# Autodesk Inventor assembly: dtandcata2
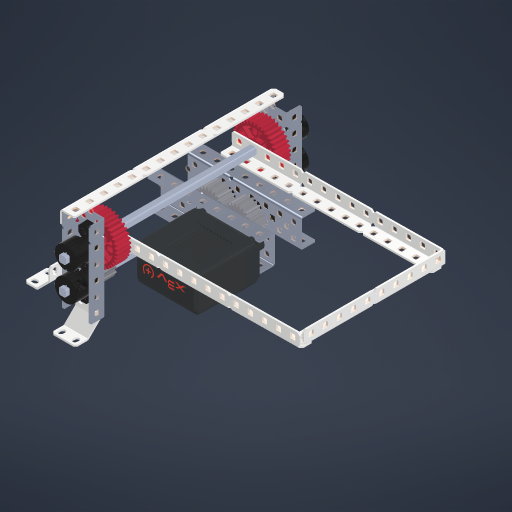
[picture p0: Inventor's stored thumbnail of the model, 512x512]
Saved by Autodesk Inventor 2024 (Build 280153000, 153)
## iProperties
Created: 2023-09-09
Part Number: dtandcata2
Document SubType Name: Assembly
Designer: macbook
Author: macbook
## Documents named in this file (22)
- \\Mac\Home\Desktop\code\1599V-VRC\Cad\Assembly\v2\dtandcata2.iam
- \\Mac\Home\Desktop\code\1599V-VRC\Cad\Assembly\v2\6wdt.iam
- \\Mac\Home\Desktop\code\1599V-VRC\Cad\Structure\Gussets\90 Angle Gusset.ipt
- \\Mac\Home\Desktop\code\1599V-VRC\Cad\Motion\Gears\HS Gear\HS 12T Gear, No Insert.iam
- \\Mac\Home\Desktop\code\1599V-VRC\Cad\Motion\Gears\HS Gear.iam
- \\Mac\Home\Desktop\code\1599V-VRC\Cad\Motion\Gears\HS Gear\HS 36T Gear, No Insert.iam
- \\Mac\Home\Desktop\code\1599V-VRC\Cad\Field\276-8354-003 Rev2_12-8 Update.ipt
- \\Mac\Home\Desktop\code\1599V-VRC\Cad\Motion\Shaft HS\HS Spacer.ipt
- \\Mac\Home\Desktop\code\1599V-VRC\Cad\Field\276-8354-260 Rev2.iam
- \\Mac\Home\Desktop\code\1599V-VRC\Cad\Structure\C Channel\Steel 1x2x1\Steel C 1x2x1x8.ipt
- \\Mac\Home\Desktop\code\1599V-VRC\Cad\Electronics\Motors with Screws\AluM-StarS_MIR5.iam
- \\Mac\Home\Desktop\code\1599V-VRC\Cad\Motion\Gears\HS Gear\HS 24T Gear, No Insert.iam
- \\Mac\Home\Desktop\code\1599V-VRC\Cad\Motion\Shaft HS\HS Spacer\HSpacer .2500.ipt
- \\Mac\Home\Desktop\code\1599V-VRC\Cad\Assembly\v2\HS Bearing Flat.ipt
- \\Mac\Home\Desktop\code\1599V-VRC\Cad\Motion\Shaft HS\HS Bearing Flat.ipt
- \\Mac\Home\Desktop\code\1599V-VRC\Cad\Motion\Shaft HS\HS Shaft Collar.ipt
- \\Mac\Home\Desktop\code\1599V-VRC\Cad\Motion\Shaft HS\Shaft HS.ipt
- \\Mac\Home\Desktop\code\1599V-VRC\Cad\Motion\Shaft HS\Shaft HS\Shaft HS 8.5 in.ipt
- \\Mac\Home\Desktop\code\1599V-VRC\Cad\Motion\Shaft HS\HS Spacer\HSpacer .1250.ipt
- \\Mac\Home\Desktop\code\1599V-VRC\Cad\Structure\Angle\Aluminum\1x1\Alu Angle 1x1x15.ipt
- \\Mac\Home\Desktop\code\1599V-VRC\Cad\Structure\Angle\Aluminum\1x1\Alu Angle 1x1x10.ipt
- \\Mac\Home\Desktop\code\1599V-VRC\Cad\Structure\C Channel\Steel 1x2x1\Steel C 1x2x1x6.ipt
## Components (42 placed, 17 different names)
1. 6wdt:1 [sub-assembly] — Mate:2, Flush:1, Mate:5, Mate:7, Mate:9, Insert:44, Insert:45, Insert:46, Insert:47
2. 90 Angle Gusset:1 — Mate:2, Flush:1
3. 90 Angle Gusset:3 — Mate:5
4. 276-8354-003 Rev2_12-8 Update:1
5. 276-8354-260 Rev2:1 [sub-assembly]
6. Steel C 1x2x1x6:1 — Insert:49
7. 90 Angle Gusset:4 — Mate:7
8. Steel C 1x2x1x8:1 — Insert:11, Insert:12, Insert:14, Insert:15, Insert:17, Insert:18, Insert:22, Insert:46, Insert:47
9. Steel C 1x2x1x8:2 — Insert:9, Insert:10, Insert:16, Insert:44, Insert:45
10. AluM-StarS_MIR5:1 [sub-assembly] — Insert:9, Insert:10
11. HS 24T Gear, No Insert:3 [sub-assembly] — Insert:11
12. HS 24T Gear, No Insert:4 [sub-assembly] — Insert:12, Insert:13
13. HSpacer .2500:1 — Insert:13
14. HSpacer .2500:2 — Insert:14
15. HSpacer .2500:3 — Insert:15
16. HSpacer .2500:4 — Insert:16
17. HS Bearing Flat:1 — Insert:17, Insert:18
18. Steel C 1x2x1x6:2
19. HS 36T Gear, No Insert:5 [sub-assembly] — Insert:33, Insert:42, Insert:43
20. 90 Angle Gusset:5 — Mate:9
21. HS Bearing Flat:2 — Insert:22
22. HS Bearing Flat:3 — Insert:31
23. HS Bearing Flat:4 — Insert:30
24. HS Bearing Flat:5 — Insert:28
25. HS Bearing Flat:6 — Insert:29
26. HS Shaft Collar:1 — Insert:28, Flush:2, Cylindrical:1
27. HS Shaft Collar:2 — Insert:29, Flush:3, Cylindrical:2
28. HS Shaft Collar:3 — Insert:30
29. HS Shaft Collar:4 — Insert:31
30. Shaft HS 8.5 in:1 — Flush:2, Cylindrical:1
31. Shaft HS 8.5 in:2 — Flush:3, Cylindrical:2
32. HSpacer .1250:5 — Insert:33
33. HS 12T Gear, No Insert:7 [sub-assembly] — Insert:34
34. HSpacer .1250:6 — Insert:34
35. HS 36T Gear, No Insert:8 [sub-assembly] — Insert:40, Insert:41
36. HSpacer .1250:7
37. HS 12T Gear, No Insert:9 [sub-assembly]
38. HSpacer .1250:8
39. Alu Angle 1x1x15:1 — Insert:40, Insert:41, Insert:48
40. Alu Angle 1x1x15:2 — Insert:42, Insert:43, Angle:2
41. Alu Angle 1x1x10:1 — Insert:48, Angle:2
42. Alu Angle 1x1x15:3 — Insert:49
## Relationships (53: Insert 40, Mate 6, Flush 3, Angle 2, CylindricalJoint 2)
- Mate:2: 6wdt:1 ↔ 90 Angle Gusset:1
- Flush:1: 6wdt:1 ↔ 90 Angle Gusset:1
- Mate:5: 6wdt:1 ↔ 90 Angle Gusset:3
- [Insert]: 6wdt:1 ↔ Steel C 1x2x1x6:1
- [Angle] (180 deg): 90 Angle Gusset:3 ↔ Steel C 1x2x1x6:1
- [Mate]: Steel C 1x2x1x6:1 ↔ 90 Angle Gusset:4
- Mate:7: 6wdt:1 ↔ 90 Angle Gusset:4
- Insert:9: Steel C 1x2x1x8:2 ↔ AluM-StarS_MIR5:1
- Insert:10: Steel C 1x2x1x8:2 ↔ AluM-StarS_MIR5:1
- Insert:11 (6.35 mm): Steel C 1x2x1x8:1 ↔ HS 24T Gear, No Insert:3
- Insert:12 (6.35 mm): Steel C 1x2x1x8:1 ↔ HS 24T Gear, No Insert:4
- Insert:13: HS 24T Gear, No Insert:4 ↔ HSpacer .2500:1
- Insert:14: Steel C 1x2x1x8:1 ↔ HSpacer .2500:2
- Insert:15: Steel C 1x2x1x8:1 ↔ HSpacer .2500:3
- Insert:16: Steel C 1x2x1x8:2 ↔ HSpacer .2500:4
- Insert:17: Steel C 1x2x1x8:1 ↔ HS Bearing Flat:1
- Insert:18: Steel C 1x2x1x8:1 ↔ HS Bearing Flat:1
- [Insert]: 6wdt:1 ↔ Steel C 1x2x1x6:2
- [Mate]: Steel C 1x2x1x6:2 ↔ 90 Angle Gusset:5
- Mate:9: 6wdt:1 ↔ 90 Angle Gusset:5
- Insert:22: Steel C 1x2x1x8:1 ↔ HS Bearing Flat:2
- [Insert]: Steel C 1x2x1x6:1 ↔ HS Bearing Flat:3
- [Insert]: Steel C 1x2x1x6:1 ↔ HS Bearing Flat:3
- [Insert]: Steel C 1x2x1x6:1 ↔ HS Bearing Flat:4
- [Insert]: Steel C 1x2x1x6:2 ↔ HS Bearing Flat:5
- [Insert]: Steel C 1x2x1x6:2 ↔ HS Bearing Flat:6
- Insert:28: HS Bearing Flat:5 ↔ HS Shaft Collar:1
- Insert:29: HS Bearing Flat:6 ↔ HS Shaft Collar:2
- Insert:30: HS Bearing Flat:4 ↔ HS Shaft Collar:3
- Insert:31: HS Bearing Flat:3 ↔ HS Shaft Collar:4
- Flush:2 (-3.048 mm): HS Shaft Collar:1 ↔ Shaft HS 8.5 in:1
- Flush:3 (-3.048 mm): HS Shaft Collar:2 ↔ Shaft HS 8.5 in:2
- Cylindrical:1: HS Shaft Collar:1 ↔ Shaft HS 8.5 in:1
- Cylindrical:2: HS Shaft Collar:2 ↔ Shaft HS 8.5 in:2
- [Insert]: Steel C 1x2x1x6:2 ↔ HSpacer .1250:5
- Insert:33: HS 36T Gear, No Insert:5 ↔ HSpacer .1250:5
- Insert:34: HS 12T Gear, No Insert:7 ↔ HSpacer .1250:6
- [Insert]: Steel C 1x2x1x6:2 ↔ HSpacer .1250:6
- [Insert]: HS 36T Gear, No Insert:8 ↔ HSpacer .1250:7
- [Insert]: HS 12T Gear, No Insert:9 ↔ HSpacer .1250:8
- [Insert]: Steel C 1x2x1x6:1 ↔ HSpacer .1250:8
- [Insert]: Steel C 1x2x1x6:1 ↔ HSpacer .1250:7
- Insert:40: HS 36T Gear, No Insert:8 ↔ Alu Angle 1x1x15:1
- Insert:41: HS 36T Gear, No Insert:8 ↔ Alu Angle 1x1x15:1
- Insert:42: HS 36T Gear, No Insert:5 ↔ Alu Angle 1x1x15:2
- Insert:43: HS 36T Gear, No Insert:5 ↔ Alu Angle 1x1x15:2
- Insert:44: 6wdt:1 ↔ Steel C 1x2x1x8:2
- Insert:45: 6wdt:1 ↔ Steel C 1x2x1x8:2
- Insert:46: 6wdt:1 ↔ Steel C 1x2x1x8:1
- Insert:47: 6wdt:1 ↔ Steel C 1x2x1x8:1
- Insert:48: Alu Angle 1x1x15:1 ↔ Alu Angle 1x1x10:1
- Angle:2 (0 deg): Alu Angle 1x1x15:2 ↔ Alu Angle 1x1x10:1
- Insert:49: Steel C 1x2x1x6:1 ↔ Alu Angle 1x1x15:3
## Named parameters: d113_d110 = 0 mm, d114_d111 = 0 mm
